# Autodesk Inventor assembly: Amplifier Assembly
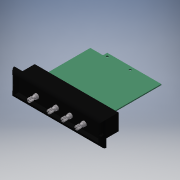
[picture p0: Inventor's stored thumbnail of the model, 180x180]
Saved by Autodesk Inventor 2017 (Build 210142000, 142)
## iProperties
Created: 2019-01-31
Part Number: Amplifier Assembly
Document SubType Name: Assembly
Designer: Mitch
Author: Mitch
## Documents named in this file (3)
- E:\Youtube Channel\Pojects\Bluetooth Speaker\MECH\Amplifier Assembly.iam
- E:\Youtube Channel\Pojects\Bluetooth Speaker\MECH\Bessel.ipt
- E:\Youtube Channel\Pojects\Bluetooth Speaker\MECH\PCB_Assembly.iam
## Components (2 placed, 2 different names)
1. Bessel:1 — Mate:2, Mate:3, Mate:4
2. PCB_Assembly:1 [sub-assembly] — Mate:2, Mate:3, Mate:4
## Relationships (3: Mate 3)
- Mate:2: Bessel:1 ↔ PCB_Assembly:1
- Mate:3 (3.175 mm): Bessel:1 ↔ PCB_Assembly:1
- Mate:4 (12.065 mm): Bessel:1 ↔ PCB_Assembly:1
